# Autodesk Inventor assembly: Собранная Мясорубка
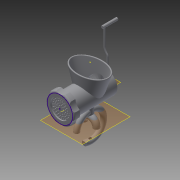
[picture p0: Inventor's stored thumbnail of the model, 180x180]
Saved by Autodesk Inventor 2014 SP1 (Build 180222100, 222)
## iProperties
Created: 2023-07-20
Part Number: Собранная Мясорубка
Document SubType Name: Assembly
Designer: 1.507-10
Author: 1.507-10
## Documents named in this file (7)
- C:\Users\Personal Computer\Desktop\SKGMI\MyPractice\Инвентор\лабораторная работа №4\Собранная Мясорубка.iam
- C:\Users\Personal Computer\Desktop\SKGMI\MyPractice\Инвентор\лабораторная работа №4\Крышка.ipt
- C:\Users\Personal Computer\Desktop\SKGMI\MyPractice\Инвентор\лабораторная работа №4\Матрица.ipt
- C:\Users\Personal Computer\Desktop\SKGMI\MyPractice\Инвентор\лабораторная работа №4\Нож.ipt
- C:\Users\Personal Computer\Desktop\SKGMI\MyPractice\Инвентор\лабораторная работа №4\Рукоять.ipt
- C:\Users\Personal Computer\Desktop\SKGMI\MyPractice\Инвентор\лабораторная работа №4\Шнек.ipt
- C:\Users\Personal Computer\Desktop\SKGMI\MyPractice\Инвентор\лабораторная работа №4\Корпус.ipt
## Components (6 placed, 6 different names)
1. Крышка:1 — Вращательный:2
2. Матрица:1 — Вращательный:2, Жесткий:2
3. Нож:1 — Жесткий:1
4. Рукоять:1 — Вращательный:3
5. Шнек:1 — Жесткий:1, Вращательный:1, Жесткий:2
6. Корпус:1 — Вращательный:1, Вращательный:3
## Relationships (5: RevoluteJoint 3, WeldJoint 2)
- Жесткий:1 [WeldJoint]: Нож:1 ↔ Шнек:1
- Вращательный:1 [RevoluteJoint]: Шнек:1 ↔ Корпус:1
- Вращательный:2 [RevoluteJoint]: Крышка:1 ↔ Матрица:1
- Жесткий:2 [WeldJoint]: Матрица:1 ↔ Шнек:1
- Вращательный:3 [RevoluteJoint]: Рукоять:1 ↔ Корпус:1
